# Autodesk Inventor assembly: Assembly
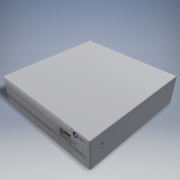
[picture p0: Inventor's stored thumbnail of the model, 180x180]
Saved by Autodesk Inventor 2018 (Build 220112000, 112)
## iProperties
Created: 2019-05-02
Part Number: Assembly
Document SubType Name: Assembly
Designer: thatg
Material: PC/ABS Plastic
Author: thatg
## Documents named in this file (7)
- C:\Users\thatg\Documents\Commodore Cube Project\Case\Assembly.iam
- C:\Users\thatg\Documents\Commodore Cube Project\Case\Tray.ipt
- C:\Users\thatg\Documents\Commodore Cube Project\Case\Dome.ipt
- C:\Users\thatg\Documents\Commodore Cube Project\Case\FloppyCover.ipt
- C:\Users\thatg\Documents\Commodore Cube Project\Case\LedCovers.ipt
- C:\Users\thatg\Documents\Commodore Cube Project\Case\Emblem.ipt
- C:\Users\thatg\Documents\Commodore Cube Project\Case\RubberFeet.ipt
## Components (6 placed, 6 different names)
1. Tray:1 — Flush:1, Flush:2, Flush:3, Flush:4, Flush:6
2. Dome:1 — Flush:1, Flush:5
3. FloppyCover:1 — Flush:2
4. LedCovers:1 — Flush:3, Flush:4
5. Emblem:1 — Flush:5
6. RubberFeet:1 — Flush:6
## Relationships (6: Flush 6)
- Flush:1: Tray:1 ↔ Dome:1
- Flush:2: Tray:1 ↔ FloppyCover:1
- Flush:3: Tray:1 ↔ LedCovers:1
- Flush:4: Tray:1 ↔ LedCovers:1
- Flush:5: Dome:1 ↔ Emblem:1
- Flush:6: Tray:1 ↔ RubberFeet:1
